# Autodesk Inventor assembly: Main_Body
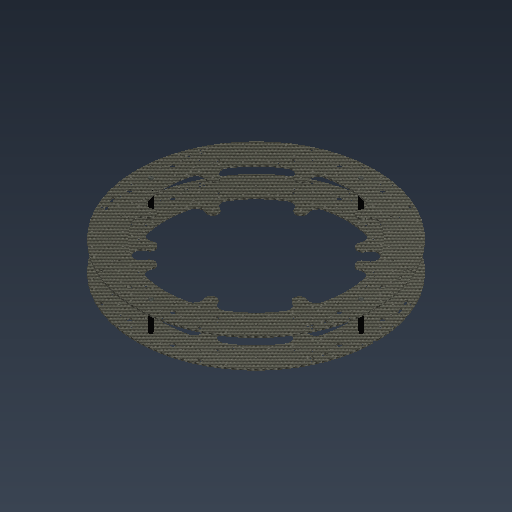
[picture p0: Inventor's stored thumbnail of the model, 512x512]
Saved by Autodesk Inventor 2024.1 (Build 281209000, 209)
## iProperties
Created: 2023-12-05
Part Number: Main_Body
Document SubType Name: Assembly
Designer: dzw04
Mass: 226.214 g
Surface Area: 1705.36 cm^2
Volume: 152.561 cm^3
Density: 1.48278 g/cm^3
Author: dzw04
## Documents named in this file (5)
- C:\Users\dzw04\Saxion\Mechatronica Lectoraat LMECH LED - Database ARG\Component_Database\SARAX\01. CAD\01. 3D_Drawing\02. Sub_Assemblies\Main_Body\Main_Body.iam
- C:\Users\dzw04\Saxion\Mechatronica Lectoraat LMECH LED - Database ARG\Component_Database\SARAX\01. CAD\01. 3D_Drawing\02. Sub_Assemblies\Main_Body\01. Parts\Body_Outer_Plate.ipt
- C:\Users\dzw04\Saxion\Mechatronica Lectoraat LMECH LED - Database ARG\Component_Database\SARAX\01. CAD\01. 3D_Drawing\01. Parts\Standoff_M3_37mm.ipt
- C:\Users\dzw04\Saxion\Mechatronica Lectoraat LMECH LED - Database ARG\Component_Database\SARAX\01. CAD\01. 3D_Drawing\01. Parts\en-US\ISO 7380-1\ISO 7380-1 - M3 x 8.ipt
- C:\Users\dzw04\Saxion\Mechatronica Lectoraat LMECH LED - Database ARG\Component_Database\SARAX\01. CAD\01. 3D_Drawing\Parameters.xlsx
## Components (14 placed, 3 different names)
1. Body_Outer_Plate:2 — Mate:1, Mate:2, Mate:3, Mate:4, Mate:5, Mate:10, Angle:1
2. Body_Outer_Plate:1 — Mate:1, Mate:2, Mate:3
3. Standoff_M3_37mm:1 — Mate:4, Mate:5, Mate:6, Mate:7, Mate:8, Mate:9
4. ISO 7380-1 M3 x 8:1 — Mate:6, Mate:9
5. ISO 7380-1 M3 x 8:2 — Mate:7, Mate:8
6. Standoff_M3_37mm:2
7. ISO 7380-1 M3 x 8:3
8. ISO 7380-1 M3 x 8:4
9. Standoff_M3_37mm:3
10. ISO 7380-1 M3 x 8:5
11. ISO 7380-1 M3 x 8:6
12. Standoff_M3_37mm:4
13. ISO 7380-1 M3 x 8:7
14. ISO 7380-1 M3 x 8:8
## Component patterns: (4 elements, first: Standoff_M3_37mm:1 + ISO 7380-1 M3 x 8:1 + ISO 7380-1 M3 x 8:2)
## Relationships (11: Mate 10, Angle 1)
- Mate:1 (37 mm): Body_Outer_Plate:2 ↔ Body_Outer_Plate:1
- Mate:2: Body_Outer_Plate:2 ↔ Body_Outer_Plate:1
- Mate:3: Body_Outer_Plate:2 ↔ Body_Outer_Plate:1
- Mate:4: Body_Outer_Plate:2 ↔ Standoff_M3_37mm:1
- Mate:5: Body_Outer_Plate:2 ↔ Standoff_M3_37mm:1
- Mate:6 (2 mm): Standoff_M3_37mm:1 ↔ ISO 7380-1 M3 x 8:1
- Mate:7 (2 mm): Standoff_M3_37mm:1 ↔ ISO 7380-1 M3 x 8:2
- Mate:8: Standoff_M3_37mm:1 ↔ ISO 7380-1 M3 x 8:2
- Mate:9: Standoff_M3_37mm:1 ↔ ISO 7380-1 M3 x 8:1
- Mate:10: Body_Outer_Plate:2
- Angle:1 (0 deg): Body_Outer_Plate:2
## Named parameters: NumberOfArms = 4, RotorToRotor = 900 mm, MountToMotorCenter = 0 mm, ArmPosition = 5 deg, LoadpipeLength = 450 mm, LandingGearHeight = 400 mm, NumberOfBatterys = 2, BatteryLength = 200 mm, BatteryWidth = 62 mm, BatteryHeight = 76 mm, ThicknessBodyOuterPlate = 2 mm, ThicknessBodyCenterPlate = 2 mm, ThicknessLegLoadpipePlate = 2 mm, ThicknessBatteryTray = 2 mm, ThicknessBatteryTopTray = 1 mm, LandingGearRod = 390 mm, LandingGearStabilityBar = 525 mm, StartAngleArm = 45 deg, MotorMountCenter = 71.5 mm
